# Autodesk Inventor assembly: Teleskop
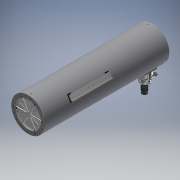
[picture p0: Inventor's stored thumbnail of the model, 180x180]
Saved by Autodesk Inventor 2019.4 (Build 234330000, 330)
## iProperties
Created: 2019-06-02
Part Number: Teleskop
Material: Ogólny
Document SubType Name: Assembly
Designer: barto
Author: barto
## Documents named in this file (19)
- F:\GOTOWY BEM\TELESKOP\Teleskop.iam
- F:\GOTOWY BEM\PRIMATYMIRROR\Gotowy.iam
- F:\GOTOWY BEM\TUBA\tuba2.ipt
- F:\GOTOWY BEM\TELESKOP\Teleskop\Design Accelerator\Połączenie gwintowe1.iam
- F:\GOTOWY BEM\TELESKOP\Teleskop\Design Accelerator\Połączenie gwintowe2.iam
- F:\GOTOWY BEM\TELESKOP\Teleskop\Design Accelerator\Połączenie gwintowe4.iam
- F:\GOTOWY BEM\TELESKOP\Teleskop\Design Accelerator\Połączenie gwintowe5.iam
- C:\Users\barto\OneDrive\Dokumenty\Inventor\Content Center Files\R2019\pl-PL\ISO 4035(2)\ISO 4035 - M3 - ISO.ipt
- F:\GOTOWY BEM\Złożenie tuba\Zespół14.iam
- F:\GOTOWY BEM\SECONDARYMIRROR2\Zespół1.iam
- F:\GOTOWY BEM\Wyciąg\wyciag.iam
- F:\GOTOWY BEM\TELESKOP\Teleskop\Design Accelerator\Połączenie gwintowe3.iam
- F:\GOTOWY BEM\TELESKOP\Teleskop\Design Accelerator\Połączenie gwintowe6.iam
- F:\GOTOWY BEM\Podkładka\podkladka2.ipt
- C:\Users\barto\OneDrive\Dokumenty\Inventor\Content Center Files\R2019\pl-PL\ISO 4035(2)\ISO 4035 - M4 - ISO.ipt
- F:\GOTOWY BEM\TELESKOP\Teleskop\Design Accelerator\Połączenie gwintowe13.iam
- F:\GOTOWY BEM\TELESKOP\Teleskop\Design Accelerator\Połączenie gwintowe14.iam
- F:\GOTOWY BEM\TELESKOP\Teleskop\Design Accelerator\Połączenie gwintowe15.iam
- F:\GOTOWY BEM\TELESKOP\Teleskop\Design Accelerator\Połączenie gwintowe16.iam
## Components (35 placed, 9 different names)
1. Gotowy:1 [sub-assembly] — Zestawiające:1, Zestawiające:2, Zestawiające:3, Zestawiające:4, Zestawiające:5, Zestawiające:6
2. tuba2:1 — Zestawiające:1, Zestawiające:2, Zestawiające:3, Zestawiające:7, Zestawiające:20, Zestawiające:21, Zestawiające:25, Zestawiające:26, Zestawiające:31, Zestawiające:32, Zestawiające:33, Zestawiające:34, Zestawiające:35, Zestawiające:36
3. Zespół1:1 [sub-assembly] — Zestawiające:20, Zestawiające:22
4. Zespół14:1 [sub-assembly] — Zestawiające:25, Zestawiające:26, Zestawiające:27, Zestawiające:28, Zestawiające:29, Zestawiające:30
5. Połączenie gwintowe:13 [sub-assembly] — Zestawiające:27, Zestawiające:28
6. Połączenie gwintowe:14 [sub-assembly] — Zestawiające:29, Zestawiające:30
7. wyciag:1 [sub-assembly] — Zestawiające:31, Zestawiające:32, Zestawiające:51, Zestawiające:52, Zestawiające:53, Zestawiające:54, Zestawiające:55, Zestawiające:56, Zestawiające:57, Zestawiające:58
8. podkladka2:1 — Zestawiające:33, Zestawiające:34, Zestawiające:47, Zestawiające:48
9. podkladka2:2 — Zestawiające:35, Zestawiające:36, Zestawiające:49, Zestawiające:50
10. ISO 4035 M4:1 — Zestawiające:48
11. ISO 4035 M4:2 — Zestawiające:47
12. ISO 4035 M4:3 — Zestawiające:49
13. ISO 4035 M4:4 — Zestawiające:50
14. Połączenie gwintowe:15 [sub-assembly] — Zestawiające:51, Zestawiające:52
15. Połączenie gwintowe:16 [sub-assembly] — Zestawiające:53, Zestawiające:54
16. Połączenie gwintowe:17 [sub-assembly] — Zestawiające:55, Zestawiające:56
17. Połączenie gwintowe:18 [sub-assembly] — Zestawiające:57, Zestawiające:58
18. Połączenie gwintowe:2 [sub-assembly] — Zestawiające:6, Zestawiające:7
19. Połączenie gwintowe:1 [sub-assembly] — Zestawiające:4, Zestawiające:5
20. Połączenie gwintowe:3 [sub-assembly]
21. Połączenie gwintowe:4 [sub-assembly]
22. Połączenie gwintowe:5 [sub-assembly]
23. Połączenie gwintowe:6 [sub-assembly]
24. Połączenie gwintowe:7 [sub-assembly] — Zestawiające:14
25. Połączenie gwintowe:8 [sub-assembly] — Zestawiające:15
26. ISO 4035 M3:1 — Zestawiające:14
27. ISO 4035 M3:2 — Zestawiające:15
28. Połączenie gwintowe:9 [sub-assembly]
29. Połączenie gwintowe:10 [sub-assembly]
30. ISO 4035 M3:3
31. ISO 4035 M3:4
32. Połączenie gwintowe:11 [sub-assembly]
33. Połączenie gwintowe:12 [sub-assembly]
34. ISO 4035 M3:5
35. ISO 4035 M3:6
## Component patterns: (3 elements, first: Połączenie gwintowe:2 + Połączenie gwintowe:1), (3 elements, first: Połączenie gwintowe:7 + Połączenie gwintowe:8 + ISO 4035 M3:1 + ISO 4035 M3:2)
## Relationships (36: Mate 36)
- Zestawiające:1 [Mate]: Gotowy:1 ↔ tuba2:1
- Zestawiające:2 [Mate]: Gotowy:1 ↔ tuba2:1
- Zestawiające:3 [Mate]: Gotowy:1 ↔ tuba2:1
- Zestawiające:4 [Mate] (3.5 mm): Gotowy:1 ↔ Połączenie gwintowe:1
- Zestawiające:5 [Mate]: Gotowy:1 ↔ Połączenie gwintowe:1
- Zestawiające:6 [Mate] (3.5 mm): Gotowy:1 ↔ Połączenie gwintowe:2
- Zestawiające:7 [Mate]: tuba2:1 ↔ Połączenie gwintowe:2
- Zestawiające:14 [Mate]: Połączenie gwintowe:7 ↔ ISO 4035 M3:1
- Zestawiające:15 [Mate]: Połączenie gwintowe:8 ↔ ISO 4035 M3:2
- Zestawiające:20 [Mate]: tuba2:1 ↔ Zespół1:1
- Zestawiające:21 [Mate]: tuba2:1
- Zestawiające:22 [Mate]: Zespół1:1
- Zestawiające:25 [Mate]: tuba2:1 ↔ Zespół14:1
- Zestawiające:26 [Mate]: tuba2:1 ↔ Zespół14:1
- Zestawiające:27 [Mate] (14 mm): Zespół14:1 ↔ Połączenie gwintowe:13
- Zestawiające:28 [Mate]: Zespół14:1 ↔ Połączenie gwintowe:13
- Zestawiające:29 [Mate] (14 mm): Zespół14:1 ↔ Połączenie gwintowe:14
- Zestawiające:30 [Mate]: Zespół14:1 ↔ Połączenie gwintowe:14
- Zestawiające:31 [Mate]: tuba2:1 ↔ wyciag:1
- Zestawiające:32 [Mate]: tuba2:1 ↔ wyciag:1
- Zestawiające:33 [Mate]: tuba2:1 ↔ podkladka2:1
- Zestawiające:34 [Mate]: tuba2:1 ↔ podkladka2:1
- Zestawiające:35 [Mate]: tuba2:1 ↔ podkladka2:2
- Zestawiające:36 [Mate]: tuba2:1 ↔ podkladka2:2
- Zestawiające:47 [Mate]: podkladka2:1 ↔ ISO 4035 M4:2
- Zestawiające:48 [Mate]: podkladka2:1 ↔ ISO 4035 M4:1
- Zestawiające:49 [Mate]: podkladka2:2 ↔ ISO 4035 M4:3
- Zestawiające:50 [Mate]: podkladka2:2 ↔ ISO 4035 M4:4
- Zestawiające:51 [Mate]: wyciag:1 ↔ Połączenie gwintowe:15
- Zestawiające:52 [Mate]: wyciag:1 ↔ Połączenie gwintowe:15
- Zestawiające:53 [Mate]: wyciag:1 ↔ Połączenie gwintowe:16
- Zestawiające:54 [Mate]: wyciag:1 ↔ Połączenie gwintowe:16
- Zestawiające:55 [Mate]: wyciag:1 ↔ Połączenie gwintowe:17
- Zestawiające:56 [Mate]: wyciag:1 ↔ Połączenie gwintowe:17
- Zestawiające:57 [Mate]: wyciag:1 ↔ Połączenie gwintowe:18
- Zestawiające:58 [Mate]: wyciag:1 ↔ Połączenie gwintowe:18
